# Autodesk Inventor assembly: Baugruppe1
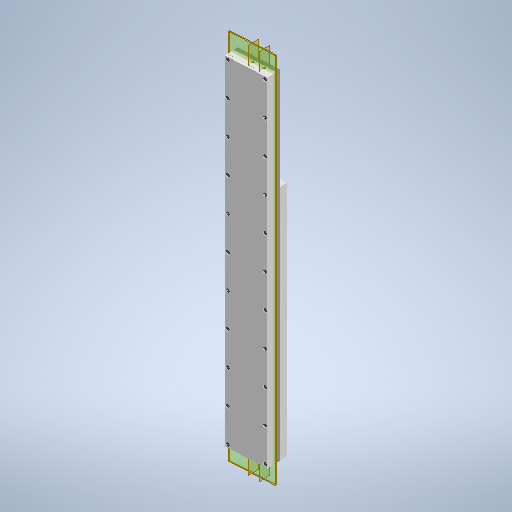
[picture p0: Inventor's stored thumbnail of the model, 512x512]
Saved by Autodesk Inventor 2025.2 (Build 292293000, 293)
## iProperties
Created: 2024-12-17
Part Number: Baugruppe1
Document SubType Name: Assembly
Designer: gorenfl4
Author: gorenfl4
## Documents named in this file (15)
- \\dfs\physik\home\gorenfl4\Desktop\MPPT_MR_GIT\Baugruppe1.iam
- \\dfs\physik\home\gorenfl4\Desktop\MPPT_MR_GIT\Bauteil5.ipt
- \\dfs\physik\home\gorenfl4\Desktop\MPPT_MR_GIT\Bauteil6.ipt
- \\dfs\physik\home\gorenfl4\Desktop\MPPT_MR_GIT\Unterer_Deckel.ipt
- \\dfs\physik\home\gorenfl4\Desktop\MPPT_MR_GIT\Maske.ipt
- \\dfs\physik\home\gorenfl4\Desktop\MPPT_MR_GIT\Bauteil4.ipt
- \\dfs\physik\home\gorenfl4\Desktop\MPPT_MR_GIT\DIN EN ISO 4762 - M2 x 3.ipt
- \\dfs\physik\home\gorenfl4\Desktop\MPPT_MR_GIT\chuck_v1.ipt
- \\dfs\physik\home\gorenfl4\Desktop\MPPT_MR_GIT\DIN EN ISO 2338 - 3 h8 x 16.ipt
- \\dfs\physik\home\gorenfl4\Desktop\MPPT_MR_GIT\DIN EN ISO 4762 - M3 x 5.ipt
- \\dfs\physik\home\gorenfl4\Desktop\MPPT_MR_GIT\DIN EN ISO 7046-2 Z - M2.5x10 - 8.8 - Z1.ipt
- \\dfs\physik\home\gorenfl4\Desktop\MPPT_MR_GIT\DIN EN ISO 4762 - M3 x 10.ipt
- \\dfs\physik\home\gorenfl4\Desktop\MPPT_MR_GIT\DIN EN ISO 4762 - M3 x 20.ipt
- \\dfs\physik\home\gorenfl4\Desktop\MPPT_MR_GIT\Glassubstrat_25x25x2,2.ipt
- \\dfs\physik\home\gorenfl4\Desktop\MPPT_MR_GIT\Glasscheibe.ipt
## Components (102 placed, 14 different names)
1. baseplate — Passend:7, Passend:8, Passend:9, Passend:26, Passend:27, Passend:28, Passend:64, Passend:65, Passend:66, Passend:67, Fluchtend:1, Fluchtend:2, Passend:70, Passend:77, Passend:78, Passend:79, Fluchtend:7, Passend:82, Passend:83, Passend:86, Passend:88, Passend:90
2. alignment frame — Passend:7, Passend:8, Passend:9, Passend:62, Passend:63, Fluchtend:1, Fluchtend:2, Passend:80, Fluchtend:8, Passend:81, Passend:84, Passend:87, Passend:91, Passend:92, Passend:131
3. bottom cover — Passend:26, Passend:27, Passend:28, Passend:64, Passend:65, Passend:66, Passend:67, Passend:85
4. mask — Passend:62, Passend:63, Passend:74, Passend:75, Einfügen:8
5. chuck_v1:2 — Passend:77, Passend:78, Passend:79
6. upper cover — Fluchtend:7, Passend:80, Fluchtend:8, Passend:89, Passend:93, Passend:94, Passend:95
7. DIN EN ISO 2338 3 h8 x 16:1 — Passend:81, Passend:82
8. DIN EN ISO 4762 M3 x 5:1 — Passend:83, Passend:84
9. substrate 25x25 — Passend:90, Passend:91, Passend:92
10. glass — Passend:93, Passend:94, Passend:95
11. DIN EN ISO 4762 M2 x 3:1 — Passend:74, Passend:75
12. DIN EN ISO 4762 M2 x 3:2
13. DIN EN ISO 4762 M2 x 3:3
14. DIN EN ISO 4762 M2 x 3:4
15. DIN EN ISO 4762 M2 x 3:5
16. DIN EN ISO 4762 M2 x 3:6
17. DIN EN ISO 4762 M2 x 3:7
18. DIN EN ISO 4762 M2 x 3:8
19. DIN EN ISO 4762 M2 x 3:9
20. DIN EN ISO 4762 M2 x 3:10
21. DIN EN ISO 4762 M2 x 3:11 — Passend:131
22. DIN EN ISO 4762 M2 x 3:12 — Einfügen:8
23. DIN EN ISO 4762 M2 x 3:13
24. DIN EN ISO 4762 M2 x 3:14
25. DIN EN ISO 4762 M2 x 3:15
26. DIN EN ISO 4762 M2 x 3:16
27. DIN EN ISO 4762 M2 x 3:17
28. DIN EN ISO 4762 M2 x 3:18
29. DIN EN ISO 4762 M2 x 3:19
30. DIN EN ISO 4762 M2 x 3:20
31. DIN EN ISO 4762 M2 x 3:21
32. DIN EN ISO 4762 M2 x 3:22
33. DIN EN ISO 7046-2 Z M2.5x10 - 8.8 - Z1:1 — Passend:85
34. DIN EN ISO 7046-2 Z M2.5x10 - 8.8 - Z1:2
35. DIN EN ISO 7046-2 Z M2.5x10 - 8.8 - Z1:3
36. DIN EN ISO 7046-2 Z M2.5x10 - 8.8 - Z1:4
37. DIN EN ISO 7046-2 Z M2.5x10 - 8.8 - Z1:5
38. DIN EN ISO 7046-2 Z M2.5x10 - 8.8 - Z1:6
39. DIN EN ISO 7046-2 Z M2.5x10 - 8.8 - Z1:7
40. DIN EN ISO 7046-2 Z M2.5x10 - 8.8 - Z1:8
41. DIN EN ISO 7046-2 Z M2.5x10 - 8.8 - Z1:9
42. DIN EN ISO 7046-2 Z M2.5x10 - 8.8 - Z1:10
43. DIN EN ISO 7046-2 Z M2.5x10 - 8.8 - Z1:11
44. DIN EN ISO 7046-2 Z M2.5x10 - 8.8 - Z1:12
45. DIN EN ISO 7046-2 Z M2.5x10 - 8.8 - Z1:13
46. DIN EN ISO 7046-2 Z M2.5x10 - 8.8 - Z1:14
47. DIN EN ISO 7046-2 Z M2.5x10 - 8.8 - Z1:15
48. DIN EN ISO 7046-2 Z M2.5x10 - 8.8 - Z1:16
49. DIN EN ISO 7046-2 Z M2.5x10 - 8.8 - Z1:17
50. DIN EN ISO 7046-2 Z M2.5x10 - 8.8 - Z1:18
51. DIN EN ISO 7046-2 Z M2.5x10 - 8.8 - Z1:19
52. DIN EN ISO 7046-2 Z M2.5x10 - 8.8 - Z1:20
53. DIN EN ISO 7046-2 Z M2.5x10 - 8.8 - Z1:21
54. DIN EN ISO 7046-2 Z M2.5x10 - 8.8 - Z1:22
55. DIN EN ISO 4762 M3 x 10:1 — Passend:86, Passend:87
56. DIN EN ISO 4762 M3 x 10:2
57. DIN EN ISO 4762 M3 x 10:3
58. DIN EN ISO 4762 M3 x 10:4
59. DIN EN ISO 4762 M3 x 10:5
60. DIN EN ISO 4762 M3 x 10:6
61. DIN EN ISO 4762 M3 x 10:7
62. DIN EN ISO 4762 M3 x 10:8
63. DIN EN ISO 4762 M3 x 10:9
64. DIN EN ISO 4762 M3 x 10:10
65. DIN EN ISO 4762 M3 x 10:11
66. DIN EN ISO 4762 M3 x 10:12
67. DIN EN ISO 4762 M3 x 10:13
68. DIN EN ISO 4762 M3 x 10:14
69. DIN EN ISO 4762 M3 x 10:15
70. DIN EN ISO 4762 M3 x 10:16
71. DIN EN ISO 4762 M3 x 10:17
72. DIN EN ISO 4762 M3 x 10:18
73. DIN EN ISO 4762 M3 x 10:19
74. DIN EN ISO 4762 M3 x 10:20
75. DIN EN ISO 4762 M3 x 20:1 — Passend:88, Passend:89
76. DIN EN ISO 4762 M3 x 20:2
77. DIN EN ISO 4762 M3 x 20:3
78. DIN EN ISO 4762 M3 x 20:4
79. DIN EN ISO 4762 M3 x 20:5
80. DIN EN ISO 4762 M3 x 20:6
81. DIN EN ISO 4762 M3 x 20:7
82. DIN EN ISO 4762 M3 x 20:8
83. DIN EN ISO 4762 M3 x 20:9
84. DIN EN ISO 4762 M3 x 20:10
85. DIN EN ISO 4762 M3 x 20:11
86. DIN EN ISO 4762 M3 x 20:12
87. DIN EN ISO 4762 M3 x 20:13
88. DIN EN ISO 4762 M3 x 20:14
89. DIN EN ISO 4762 M3 x 20:15
90. DIN EN ISO 4762 M3 x 20:16
91. DIN EN ISO 4762 M3 x 20:17
92. DIN EN ISO 4762 M3 x 20:18
93. DIN EN ISO 4762 M3 x 20:19
94. DIN EN ISO 4762 M3 x 20:20
95. DIN EN ISO 4762 M3 x 20:21
96. DIN EN ISO 4762 M3 x 20:22
97. DIN EN ISO 4762 M3 x 20:23
98. DIN EN ISO 4762 M3 x 20:24
99. DIN EN ISO 4762 M3 x 20:25
100. DIN EN ISO 4762 M3 x 20:26
101. DIN EN ISO 4762 M3 x 20:27
102. DIN EN ISO 4762 M3 x 20:28
## Component patterns: (11 elements, first: DIN EN ISO 4762 M2 x 3:1), (11 elements, first: DIN EN ISO 4762 M2 x 3:12), (22 elements, first: DIN EN ISO 7046-2 Z M2.5x10 - 8.8 - Z1:1), (20 elements, first: DIN EN ISO 4762 M3 x 10:1), (28 elements, first: DIN EN ISO 4762 M3 x 20:1)
## Relationships (41: Mate 36, Flush 4, Insert 1)
- Passend:7 [Mate]: baseplate ↔ alignment frame
- Passend:8 [Mate]: baseplate ↔ alignment frame
- Passend:9 [Mate]: baseplate ↔ alignment frame
- Passend:26 [Mate]: baseplate ↔ bottom cover
- Passend:27 [Mate]: baseplate ↔ bottom cover
- Passend:28 [Mate]: baseplate ↔ bottom cover
- Passend:62 [Mate]: alignment frame ↔ mask
- Passend:63 [Mate]: alignment frame ↔ mask
- Passend:64 [Mate]: baseplate ↔ bottom cover
- Passend:65 [Mate]: baseplate ↔ bottom cover
- Passend:66 [Mate]: baseplate ↔ bottom cover
- Passend:67 [Mate]: baseplate ↔ bottom cover
- Fluchtend:1 [Flush]: baseplate ↔ alignment frame
- Fluchtend:2 [Flush]: baseplate ↔ alignment frame
- Passend:70 [Mate]: baseplate
- Passend:74 [Mate]: mask ↔ DIN EN ISO 4762 M2 x 3:1
- Passend:75 [Mate]: mask ↔ DIN EN ISO 4762 M2 x 3:1
- Einfügen:8 [Insert]: mask ↔ DIN EN ISO 4762 M2 x 3:12
- Passend:77 [Mate]: baseplate ↔ chuck_v1:2
- Passend:78 [Mate]: baseplate ↔ chuck_v1:2
- Passend:79 [Mate]: baseplate ↔ chuck_v1:2
- Fluchtend:7 [Flush]: baseplate ↔ upper cover
- Passend:80 [Mate]: alignment frame ↔ upper cover
- Fluchtend:8 [Flush]: alignment frame ↔ upper cover
- Passend:81 [Mate]: alignment frame ↔ DIN EN ISO 2338 3 h8 x 16:1
- Passend:82 [Mate]: baseplate ↔ DIN EN ISO 2338 3 h8 x 16:1
- Passend:83 [Mate]: baseplate ↔ DIN EN ISO 4762 M3 x 5:1
- Passend:84 [Mate]: alignment frame ↔ DIN EN ISO 4762 M3 x 5:1
- Passend:85 [Mate]: bottom cover ↔ DIN EN ISO 7046-2 Z M2.5x10 - 8.8 - Z1:1
- Passend:86 [Mate]: baseplate ↔ DIN EN ISO 4762 M3 x 10:1
- Passend:87 [Mate]: alignment frame ↔ DIN EN ISO 4762 M3 x 10:1
- Passend:88 [Mate]: baseplate ↔ DIN EN ISO 4762 M3 x 20:1
- Passend:89 [Mate]: upper cover ↔ DIN EN ISO 4762 M3 x 20:1
- Passend:90 [Mate]: baseplate ↔ substrate 25x25
- Passend:91 [Mate]: alignment frame ↔ substrate 25x25
- Passend:92 [Mate]: alignment frame ↔ substrate 25x25
- Passend:93 [Mate]: upper cover ↔ glass
- Passend:94 [Mate]: upper cover ↔ glass
- Passend:95 [Mate]: upper cover ↔ glass
- Passend:110 [Mate]
- Passend:131 [Mate]: alignment frame ↔ DIN EN ISO 4762 M2 x 3:11
